# Autodesk Inventor assembly: Shaft_Sprocket_Assembly
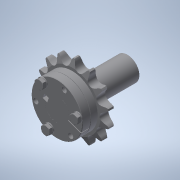
[picture p0: Inventor's stored thumbnail of the model, 180x180]
Saved by Autodesk Inventor 2021 (Build 250183000, 183)
## iProperties
Created: 2020-10-13
Part Number: Shaft_Sprocket_Assembly
Document SubType Name: Assembly
Designer: PhotonUser
Quantity: 1
Author: PhotonUser
## Documents named in this file (4)
- D:\PhotonUser\Downloads\Assembly Files-20201019T222523Z-001\Assembly Files\Shaft_Sprocket_Assembly.iam
- D:\PhotonUser\Downloads\Assembly Files-20201019T222523Z-001\Assembly Files\6086K221_QUICK-DISCONNECT BUSHING.ipt
- D:\PhotonUser\Downloads\Assembly Files-20201019T222523Z-001\Assembly Files\62375K141_QUICK-DISCONNECT BUSHING-BORE SPROCKET.ipt
- D:\PhotonUser\Downloads\Assembly Files-20201019T222523Z-001\Assembly Files\MotorShaft.ipt
## Components (3 placed, 3 different names)
1. 6086K221_QUICK-DISCONNECT BUSHING:1 — Insert:1, Insert:2, Mate:1, Flush:1, Flush:2
2. 62375K141_QUICK-DISCONNECT BUSHING-BORE SPROCKET:1 — Insert:1, Insert:2
3. MotorShaft:1 — Mate:1, Flush:1, Flush:2
## Relationships (5: Insert 2, Flush 2, Mate 1)
- Insert:1: 6086K221_QUICK-DISCONNECT BUSHING:1 ↔ 62375K141_QUICK-DISCONNECT BUSHING-BORE SPROCKET:1
- Insert:2: 6086K221_QUICK-DISCONNECT BUSHING:1 ↔ 62375K141_QUICK-DISCONNECT BUSHING-BORE SPROCKET:1
- Mate:1: 6086K221_QUICK-DISCONNECT BUSHING:1 ↔ MotorShaft:1
- Flush:1: 6086K221_QUICK-DISCONNECT BUSHING:1 ↔ MotorShaft:1
- Flush:2: 6086K221_QUICK-DISCONNECT BUSHING:1 ↔ MotorShaft:1
